# Autodesk Inventor assembly: Assembly1
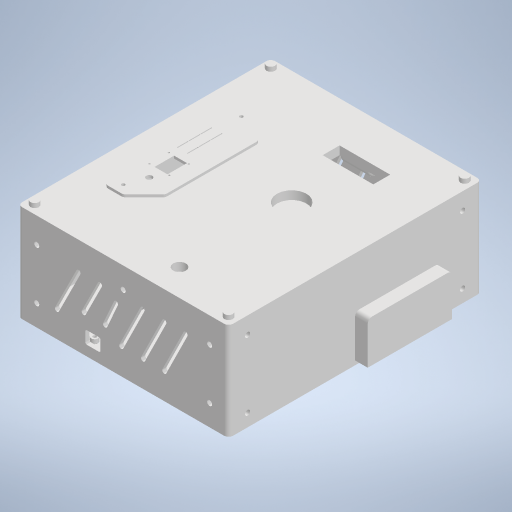
[picture p0: Inventor's stored thumbnail of the model, 512x512]
Saved by Autodesk Inventor 2024 (Build 280153000, 153)
## iProperties
Created: 2026-03-18
Part Number: Assembly1
Document SubType Name: Assembly
Designer: Acer
Author: Acer
## Documents named in this file (9)
- G:\Inne komputery\Acer (stacjonarka)\Space Team\1_Projekt_Stazowy\Podgrzewacz\github\casing_prototyping\Assembly2.iam
- G:\Inne komputery\Acer (stacjonarka)\Space Team\1_Projekt_Stazowy\Podgrzewacz\github\casing_prototyping\Bottom.ipt
- G:\Inne komputery\Acer (stacjonarka)\Space Team\1_Projekt_Stazowy\Podgrzewacz\github\casing_prototyping\legs.ipt
- G:\Inne komputery\Acer (stacjonarka)\Space Team\1_Projekt_Stazowy\Podgrzewacz\github\casing_prototyping\left_side.ipt
- G:\Inne komputery\Acer (stacjonarka)\Space Team\1_Projekt_Stazowy\Podgrzewacz\github\casing_prototyping\right_side.ipt
- G:\Inne komputery\Acer (stacjonarka)\Space Team\1_Projekt_Stazowy\Podgrzewacz\github\casing_prototyping\side_front.ipt
- G:\Inne komputery\Acer (stacjonarka)\Space Team\1_Projekt_Stazowy\Podgrzewacz\github\casing_prototyping\side_back.ipt
- G:\Inne komputery\Acer (stacjonarka)\Space Team\1_Projekt_Stazowy\Podgrzewacz\github\casing_prototyping\panel.ipt
- G:\Inne komputery\Acer (stacjonarka)\Space Team\1_Projekt_Stazowy\Podgrzewacz\github\casing_prototyping\top.ipt
## Components (11 placed, 8 different names)
1. Bottom:1 — Mate:4, Mate:5, Mate:6, Mate:7, Mate:8, Mate:9, Mate:10, Mate:11, Mate:18
2. legs:1 — Mate:6
3. legs:2 — Mate:5
4. legs:3 — Mate:4
5. legs:4 — Mate:7
6. left_side:1 — Mate:8
7. right_side:1 — Mate:9
8. side_front:1 — Mate:10
9. side_back:1 — Mate:11
10. panel:1 — Mate:12
11. top:1 — Mate:12, Mate:18
## Relationships (10: Mate 10)
- Mate:4: Bottom:1 ↔ legs:3
- Mate:5: Bottom:1 ↔ legs:2
- Mate:6: Bottom:1 ↔ legs:1
- Mate:7: Bottom:1 ↔ legs:4
- Mate:8: Bottom:1 ↔ left_side:1
- Mate:9: Bottom:1 ↔ right_side:1
- Mate:10: Bottom:1 ↔ side_front:1
- Mate:11: Bottom:1 ↔ side_back:1
- Mate:12: panel:1 ↔ top:1
- Mate:18: Bottom:1 ↔ top:1
